# Autodesk Inventor assembly: Mold Design1
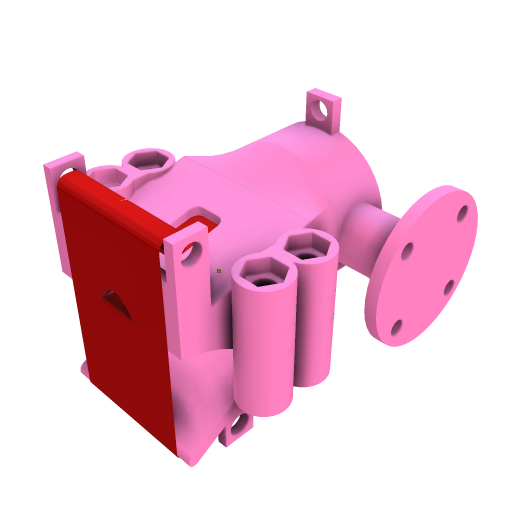
[picture p0: Inventor's stored thumbnail of the model, 512x512]
Saved by Autodesk Inventor 2024 (Build 280153000, 153)
## iProperties
Created: 2023-04-14
Part Number: Mold Design1
Document SubType Name: Assembly
Designer: ferna
Author: ferna
## Documents named in this file (4)
- C:\Users\ferna\OneDrive - Universidad Católica de Chile\Bocas\RobotFlautista\Mold Design1\Mold Design1.iam
- C:\Users\ferna\OneDrive - Universidad Católica de Chile\Bocas\RobotFlautista\nueva_boca_3 - Copy (2).ipt
- C:\Users\ferna\OneDrive - Universidad Católica de Chile\Bocas\RobotFlautista\nueva_boca_3 - Copy (3).ipt
- C:\Users\ferna\OneDrive - Universidad Católica de Chile\Bocas\RobotFlautista\nueva_boca_3 - Copy.ipt
## Components (3 placed, 3 different names)
1. nueva_boca_3 - Copy (2):1 — Mate:1, Mate:2, Mate:3, Mate:4, Mate:5, Mate:6
2. nueva_boca_3 - Copy (3):1 — Mate:4, Mate:5, Mate:6
3. nueva_boca_3 - Copy:1 — Mate:1, Mate:2, Mate:3
## Relationships (6: Mate 6)
- Mate:1: nueva_boca_3 - Copy (2):1 ↔ nueva_boca_3 - Copy:1
- Mate:2: nueva_boca_3 - Copy (2):1 ↔ nueva_boca_3 - Copy:1
- Mate:3: nueva_boca_3 - Copy (2):1 ↔ nueva_boca_3 - Copy:1
- Mate:4: nueva_boca_3 - Copy (2):1 ↔ nueva_boca_3 - Copy (3):1
- Mate:5: nueva_boca_3 - Copy (2):1 ↔ nueva_boca_3 - Copy (3):1
- Mate:6: nueva_boca_3 - Copy (2):1 ↔ nueva_boca_3 - Copy (3):1
